# Autodesk Inventor assembly: Base
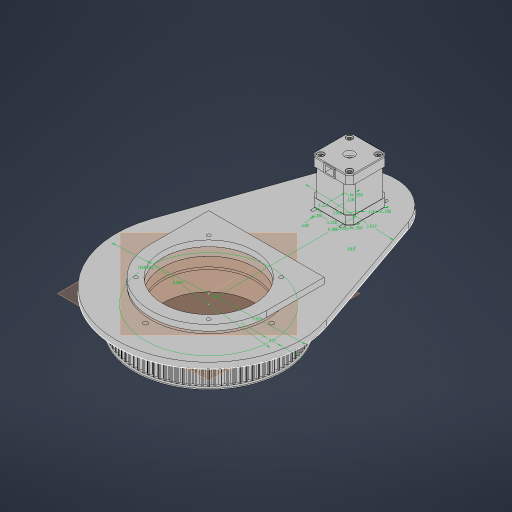
[picture p0: Inventor's stored thumbnail of the model, 512x512]
Saved by Autodesk Inventor 2024 (Build 280153000, 153)
## iProperties
Created: 2023-10-21
Part Number: Base
Document SubType Name: Assembly
Designer: range
Author: range
## Documents named in this file (7)
- C:\Users\range\CodingProjects\C-AAM\CAD\V1\Base.iam
- C:\Users\range\CodingProjects\C-AAM\CAD\V1\Parts\LazySusan.iam
- C:\Users\range\CodingProjects\C-AAM\CAD\V1\LargePitchAssembly.iam
- C:\Users\range\CodingProjects\C-AAM\CAD\V1\WCP-0562\WCP-0562.ipt
- C:\Users\range\CodingProjects\C-AAM\CAD\V1\Parts\Board.ipt
- C:\Users\range\CodingProjects\C-AAM\CAD\V1\6627T91_Stepper Motor\6627T91_Stepper Motor.ipt
- C:\Users\range\CodingProjects\C-AAM\CAD\V1\Parts\2ndAxis.iam
## Components (6 placed, 6 different names)
1. LazySusan:1 [sub-assembly] — Flush:2, Flush:3, Mate:6, Mate:7, Mate:8, Mate:11, Flush:4, Mate:12, Mate:13
2. LargePitchAssembly:1 [sub-assembly] — Mate:7, Flush:5
3. WCP-0562:1 — Mate:5, Angle:2, Flush:5
4. Board:1 — Flush:2, Flush:3, Mate:4, Mate:6, Mate:8, Mate:11, Angle:1, Mate:14
5. 6627T91_Stepper Motor:1 — Mate:4, Mate:5, Angle:1, Mate:14, Angle:2
6. 2ndAxis:1 [sub-assembly] — Flush:4, Mate:12, Mate:13
## Relationships (17: Mate 11, Flush 4, Angle 2)
- [Mate] (2.5 mm): LazySusan:1 ↔ LargePitchAssembly:1
- [Mate]: LazySusan:1 ↔ LargePitchAssembly:1
- Flush:2: LazySusan:1 ↔ Board:1
- Flush:3: LazySusan:1 ↔ Board:1
- Mate:4: Board:1 ↔ 6627T91_Stepper Motor:1
- Mate:5: WCP-0562:1 ↔ 6627T91_Stepper Motor:1
- Mate:6: LazySusan:1 ↔ Board:1
- Mate:7: LazySusan:1 ↔ LargePitchAssembly:1
- Mate:8: LazySusan:1 ↔ Board:1
- Mate:11: LazySusan:1 ↔ Board:1
- Flush:4: LazySusan:1 ↔ 2ndAxis:1
- Mate:12: LazySusan:1 ↔ 2ndAxis:1
- Mate:13: LazySusan:1 ↔ 2ndAxis:1
- Angle:1 (0 deg): Board:1 ↔ 6627T91_Stepper Motor:1
- Mate:14: Board:1 ↔ 6627T91_Stepper Motor:1
- Angle:2 (180 deg): WCP-0562:1 ↔ 6627T91_Stepper Motor:1
- Flush:5: LargePitchAssembly:1 ↔ WCP-0562:1
